# Autodesk Inventor assembly: A2017_T5_01
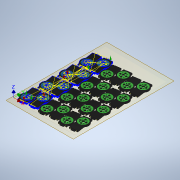
[picture p0: Inventor's stored thumbnail of the model, 180x180]
Saved by Autodesk Inventor 2022 (Build 260153000, 153)
## iProperties
Created: 2022-09-28
Part Number: A2017_T5_01
Document SubType Name: Assembly
Designer: Masato
Author: Masato
## Documents named in this file (3)
- C:\Users\6343y\ドキュメント\Inventor\SUSTAINA-OP\Cam\A2017_T5\A2017_T5_01.iam
- C:\Users\6343y\ドキュメント\Inventor\SUSTAINA-OP\Cam\DisposableBoard.ipt
- C:\Users\6343y\ドキュメント\Inventor\SUSTAINA-OP\LowerBody\Leg_joint\Leg_joint_yaw_frame.ipt
## Components (25 placed, 2 different names)
1. DisposableBoard:1 — フラッシュ:1, フラッシュ:2, フラッシュ:3, フラッシュ:4, 正接:1, メイト:3, メイト:4
2. Leg_joint_yaw_frame:1 — メイト:1, 正接:1, 正接:2, メイト:3, メイト:4, 正接:3, 正接:4
3. Leg_joint_yaw_frame:2 — メイト:2, 正接:2, 正接:3, 正接:4
4. Leg_joint_yaw_frame:3
5. Leg_joint_yaw_frame:4
6. Leg_joint_yaw_frame:5
7. Leg_joint_yaw_frame:6
8. Leg_joint_yaw_frame:7
9. Leg_joint_yaw_frame:8
10. Leg_joint_yaw_frame:9
11. Leg_joint_yaw_frame:10
12. Leg_joint_yaw_frame:11
13. Leg_joint_yaw_frame:12
14. Leg_joint_yaw_frame:13
15. Leg_joint_yaw_frame:14
16. Leg_joint_yaw_frame:15
17. Leg_joint_yaw_frame:16
18. Leg_joint_yaw_frame:17
19. Leg_joint_yaw_frame:18
20. Leg_joint_yaw_frame:19
21. Leg_joint_yaw_frame:20
22. Leg_joint_yaw_frame:21
23. Leg_joint_yaw_frame:22
24. Leg_joint_yaw_frame:23
25. Leg_joint_yaw_frame:24
## Component patterns: (12 elements, first: Leg_joint_yaw_frame:1 + Leg_joint_yaw_frame:2)
## Relationships (12: Flush 4, Mate 4, Tangent 4)
- フラッシュ:1 [Flush]: DisposableBoard:1
- フラッシュ:2 [Flush]: DisposableBoard:1
- フラッシュ:3 [Flush]: DisposableBoard:1
- フラッシュ:4 [Flush]: DisposableBoard:1
- メイト:1 [Mate]: Leg_joint_yaw_frame:1
- メイト:2 [Mate]: Leg_joint_yaw_frame:2
- 正接:1 [Tangent] (2.063 mm): DisposableBoard:1 ↔ Leg_joint_yaw_frame:1
- 正接:2 [Tangent] (2.1 mm): Leg_joint_yaw_frame:1 ↔ Leg_joint_yaw_frame:2
- メイト:3 [Mate] (-2.063 mm): DisposableBoard:1 ↔ Leg_joint_yaw_frame:1
- メイト:4 [Mate] (-2.1 mm): DisposableBoard:1 ↔ Leg_joint_yaw_frame:1
- 正接:3 [Tangent] (2.1 mm): Leg_joint_yaw_frame:1 ↔ Leg_joint_yaw_frame:2
- 正接:4 [Tangent] (2.1 mm): Leg_joint_yaw_frame:1 ↔ Leg_joint_yaw_frame:2
